# Autodesk Inventor assembly: Assembly new
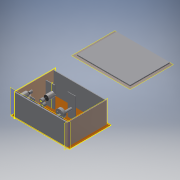
[picture p0: Inventor's stored thumbnail of the model, 180x180]
Saved by Autodesk Inventor 2019 (Build 230136000, 136)
## iProperties
Created: 2020-04-17
Part Number: Assembly new
Document SubType Name: Assembly
Designer: Pranav Naik
Author: Pranav Naik
## Documents named in this file (13)
- C:\Users\Pranav Naik\Documents\Assembly new.iam
- C:\Users\Pranav Naik\Downloads\roller3 grp17.ipt
- C:\Users\Pranav Naik\Downloads\Motor DC.ipt
- C:\Users\Pranav Naik\Downloads\roller1 grp17.ipt
- C:\Users\Pranav Naik\Documents\actual base.ipt
- C:\Users\Pranav Naik\Documents\walls.ipt
- C:\Users\Pranav Naik\Documents\Part3.ipt
- C:\Users\Pranav Naik\Documents\Part5.ipt
- C:\Users\Pranav Naik\Documents\Part6.ipt
- C:\Users\Pranav Naik\Documents\Part9.ipt
- C:\Users\Pranav Naik\Documents\Part1.ipt
- C:\Users\Pranav Naik\Documents\Part2.ipt
- C:\Users\Pranav Naik\Documents\Part4.ipt
## Components (15 placed, 12 different names)
1. roller3 grp17:1
2. Motor DC:1
3. roller1 grp17:1
4. actual base:1 — Flush:1, Flush:2, Flush:3, Flush:4, Flush:5, Flush:6, Flush:7, Flush:10, Flush:11, Flush:12, Flush:25, Flush:26
5. roller3 grp17:2
6. Motor DC:2
7. walls:1 — Flush:1, Flush:2, Flush:3, Flush:4, Flush:5, Flush:6, Flush:8, Flush:9, Flush:16, Flush:20, Flush:23, Flush:24
8. Part3:1 — Flush:7, Flush:8, Flush:9, Flush:10, Flush:11, Flush:12, Flush:13, Flush:14, Flush:21, Flush:22
9. Part5:1 — Flush:13, Flush:14, Flush:15
10. Motor DC:3
11. Part6:1 — Flush:15, Flush:16
12. Part9:1 — Flush:20
13. Part1:1 — Flush:21, Flush:22
14. Part2:1 — Flush:23, Flush:24
15. Part4:1 — Flush:25, Flush:26
## Relationships (23: Flush 23)
- Flush:1: actual base:1 ↔ walls:1
- Flush:2: actual base:1 ↔ walls:1
- Flush:3: actual base:1 ↔ walls:1
- Flush:4: actual base:1 ↔ walls:1
- Flush:5: actual base:1 ↔ walls:1
- Flush:6: actual base:1 ↔ walls:1
- Flush:7: actual base:1 ↔ Part3:1
- Flush:8: walls:1 ↔ Part3:1
- Flush:9: walls:1 ↔ Part3:1
- Flush:10: actual base:1 ↔ Part3:1
- Flush:11: actual base:1 ↔ Part3:1
- Flush:12: actual base:1 ↔ Part3:1
- Flush:13: Part3:1 ↔ Part5:1
- Flush:14: Part3:1 ↔ Part5:1
- Flush:15: Part5:1 ↔ Part6:1
- Flush:16: walls:1 ↔ Part6:1
- Flush:20: walls:1 ↔ Part9:1
- Flush:21: Part3:1 ↔ Part1:1
- Flush:22: Part3:1 ↔ Part1:1
- Flush:23: walls:1 ↔ Part2:1
- Flush:24: walls:1 ↔ Part2:1
- Flush:25: actual base:1 ↔ Part4:1
- Flush:26: actual base:1 ↔ Part4:1
